# Autodesk Inventor assembly: Weapon Disk
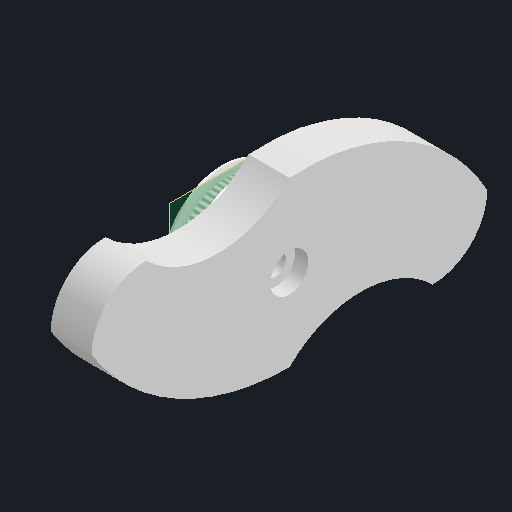
[picture p0: Inventor's stored thumbnail of the model, 512x512]
Saved by Autodesk Inventor 2026.2 (Build 302298000, 298)
## iProperties
Created: 2023-09-02
Part Number: Weapon Disk
Document SubType Name: Assembly
Designer: vandj
Author: vandj
## Documents named in this file (3)
- C:\Users\chigg\Robot_Spring_Semester\Robot_Model\07)_Weapon Assembly V5 - Horizotal Spinner.iam
- C:\Users\chigg\Robot_Spring_Semester\Robot_Model\08)_Base Weapon V5 - Horizontal Spinner.ipt
- C:\Users\chigg\Robot_Spring_Semester\Robot_Model\09)_GT2 60 Tooth Pulley.ipt
## Components (2 placed, 2 different names)
1. 08)_Base Weapon V5 - Horizontal Spinner:1 — Mate:1, Mate:2, Mate:3, Mate:4, Flush:1
2. 09)_GT2 60 Tooth Pulley:1 — Mate:1, Mate:2
## Relationships (5: Mate 4, Flush 1)
- Mate:1: 08)_Base Weapon V5 - Horizontal Spinner:1 ↔ 09)_GT2 60 Tooth Pulley:1
- Mate:2: 08)_Base Weapon V5 - Horizontal Spinner:1 ↔ 09)_GT2 60 Tooth Pulley:1
- Mate:3: 08)_Base Weapon V5 - Horizontal Spinner:1
- Mate:4: 08)_Base Weapon V5 - Horizontal Spinner:1
- Flush:1: 08)_Base Weapon V5 - Horizontal Spinner:1
